# Autodesk Inventor assembly: Shield Support
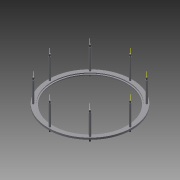
[picture p0: Inventor's stored thumbnail of the model, 180x180]
Saved by Autodesk Inventor 2015 (Build 190159000, 159)
## iProperties
Created: 2014-07-02
Part Number: Shield Support
Document SubType Name: Assembly
Designer: Aki
Author: Aki
## Documents named in this file (3)
- C:\ColdMatter\CADFiles\EDM Machine\Microwave Detection Region\Shield Support.iam
- C:\ColdMatter\CADFiles\EDM Machine\Microwave Detection Region\Shield Support Ring.ipt
- C:\ColdMatter\CADFiles\EDM Machine\Microwave Detection Region\Rod Design.ipt
## Components (9 placed, 2 different names)
1. Shield Support Ring:1 — Mate:1, Rotational:1, Rigid:1, Rigid:2, Rotational:2, Rotational:3, Rotational:4, Rotational:5, Rotational:6
2. Rod Design:1 — Rigid:1
3. Rod Design:2 — Rotational:1
4. Rod Design:3 — Rotational:6
5. Rod Design:4 — Rotational:5
6. Rod Design:5 — Rotational:4
7. Rod Design:6 — Rotational:3
8. Rod Design:7 — Rotational:2
9. Rod Design:8 — Rigid:2
## Relationships (9: RevoluteJoint 6, WeldJoint 2, Mate 1)
- Mate:1: Shield Support Ring:1
- Rotational:1 [RevoluteJoint]: Shield Support Ring:1 ↔ Rod Design:2
- Rigid:1 [WeldJoint]: Shield Support Ring:1 ↔ Rod Design:1
- Rigid:2 [WeldJoint]: Shield Support Ring:1 ↔ Rod Design:8
- Rotational:2 [RevoluteJoint]: Shield Support Ring:1 ↔ Rod Design:7
- Rotational:3 [RevoluteJoint]: Shield Support Ring:1 ↔ Rod Design:6
- Rotational:4 [RevoluteJoint]: Shield Support Ring:1 ↔ Rod Design:5
- Rotational:5 [RevoluteJoint]: Shield Support Ring:1 ↔ Rod Design:4
- Rotational:6 [RevoluteJoint]: Shield Support Ring:1 ↔ Rod Design:3
